# Autodesk Inventor assembly: assemble
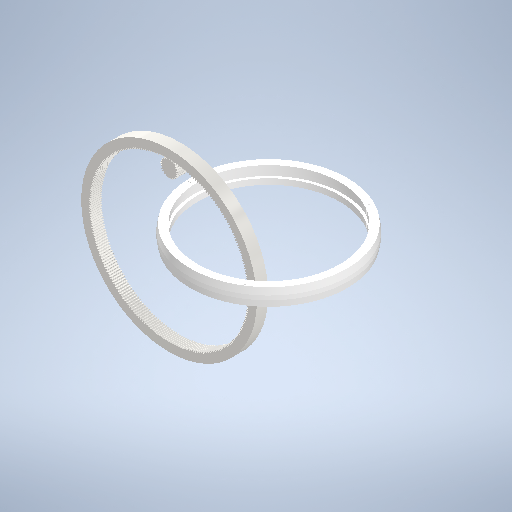
[picture p0: Inventor's stored thumbnail of the model, 512x512]
Saved by Autodesk Inventor 2025 (Build 290162000, 162)
## iProperties
Created: 2025-09-25
Part Number: assemble
Document SubType Name: Assembly
Designer: Admin
Author: Admin
## Documents named in this file (3)
- C:\Users\sum89\OneDrive\Рабочий стол\Ring\Model\assemble.iam
- C:\Users\sum89\OneDrive\Рабочий стол\Ring\Model\Inner_ring.ipt
- C:\Users\sum89\OneDrive\Рабочий стол\Ring\Model\assemble\Мастер проектирования\Цилиндрическое зубчатое зацепление1.iam
## Components (4 placed, 2 different names)
1. Inner_ring:1 — Жесткий:1
2. Inner_ring:2 — Жесткий:2
3. Inner_ring:3 — Жесткий:1, Жесткий:2
4. Цилиндрическое зубчатое зацепление:1 [sub-assembly]
## Relationships (2: WeldJoint 2)
- Жесткий:1 [WeldJoint]: Inner_ring:1 ↔ Inner_ring:3
- Жесткий:2 [WeldJoint]: Inner_ring:2 ↔ Inner_ring:3
